# Autodesk Inventor assembly: assembly
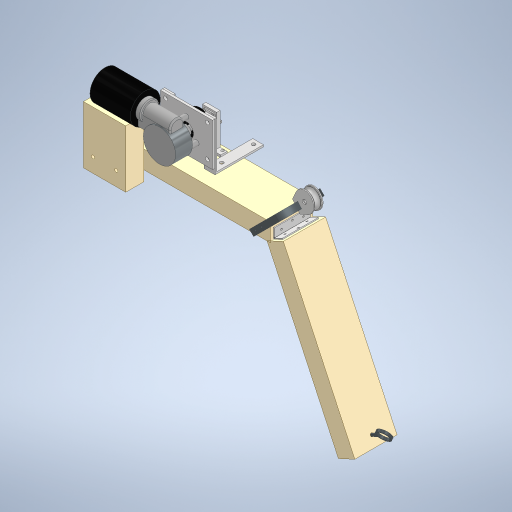
[picture p0: Inventor's stored thumbnail of the model, 512x512]
Saved by Autodesk Inventor 2024.3 (Build 283343000, 343)
## iProperties
Created: 2024-11-18
Part Number: assembly
Document SubType Name: Assembly
Designer: email
Author: email
## Documents named in this file (16)
- C:\Users\email\Desktop\Projects\Capstone\pidtest\assembly.iam
- C:\Users\email\Desktop\Projects\Capstone\pidtest\hinge.ipt
- C:\Users\email\Desktop\Projects\Capstone\pidtest\shin2x4.ipt
- C:\Users\email\Desktop\Projects\Capstone\pidtest\thigh2x4.ipt
- C:\Users\email\Desktop\Projects\Capstone\motor cad\motor.ipt
- C:\Users\email\Desktop\Projects\Capstone\pidtest\pulleybracket.ipt
- C:\Users\email\Desktop\Projects\Capstone\pidtest\hook.ipt
- C:\Users\email\Desktop\Projects\Capstone\motor cad\spool_temp.ipt
- C:\Users\email\Desktop\Projects\Capstone\pidtest\backmotormount.ipt
- C:\Users\email\Desktop\Projects\Capstone\pidtest\Lbracket.ipt
- C:\Users\email\Desktop\Projects\Capstone\pidtest\motorbracket2.ipt
- C:\Users\email\Desktop\Projects\Capstone\pidtest\pulley.ipt
- C:\Users\email\Desktop\Projects\Capstone\pidtest\pulleybearing.ipt
- C:\Users\email\Desktop\Projects\Capstone\pidtest\as5600mount.ipt
- C:\Users\email\Desktop\Projects\Capstone\pidtest\as5600.ipt
- C:\Users\email\Desktop\Projects\Capstone\pidtest\magnetholder.ipt
## Components (17 placed, 15 different names)
1. hinge:1 — Mate:1, Flush:2, Mate:33, Mate:34
2. shin2x4:1 — Mate:4, Flush:1, Mate:15, Mate:16, Mate:35
3. thigh2x4:1 — Mate:1, Flush:1, Mate:13, Mate:14, Mate:20, Mate:22, Mate:25, Mate:26, Flush:2, Mate:33, Mate:36, Mate:40, Mate:41, Mate:42, Mate:46, Mate:55, Mate:56
4. hinge:2 — Mate:4, Mate:34, Mate:35
5. motor:1 — Mate:17, Mate:18, Mate:19, Mate:30, Mate:31, Mate:32
6. pulleybracket:1 — Mate:13, Mate:14, Mate:36, Mate:37
7. hook:1 — Mate:15, Mate:16
8. spool_temp:1 — Mate:17, Mate:18, Mate:19, Mate:52, Mate:53, Mate:54
9. backmotormount:1 — Mate:20, Mate:22, Mate:40
10. Lbracket:1 — Mate:26, Mate:42, Mate:43
11. Lbracket:2 — Mate:25, Mate:41, Mate:44, Mate:45
12. motorbracket2:1 — Mate:30, Mate:31, Mate:32, Mate:43, Mate:44, Mate:45
13. pulley:1 — Mate:37, Mate:38, Mate:39
14. pulleybearing:1 — Mate:38, Mate:39
15. as5600mount:1 — Mate:46, Mate:49, Mate:50, Mate:51, Mate:55, Mate:56
16. as5600:1 — Mate:49, Mate:50, Mate:51
17. magnetholder:1 — Mate:52, Mate:53, Mate:54
## Relationships (40: Mate 38, Flush 2)
- Mate:1: hinge:1 ↔ thigh2x4:1
- Mate:4: shin2x4:1 ↔ hinge:2
- Flush:1: shin2x4:1 ↔ thigh2x4:1
- Mate:13: thigh2x4:1 ↔ pulleybracket:1
- Mate:14: thigh2x4:1 ↔ pulleybracket:1
- Mate:15: shin2x4:1 ↔ hook:1
- Mate:16 (-12.7 mm): shin2x4:1 ↔ hook:1
- Mate:17: motor:1 ↔ spool_temp:1
- Mate:18: motor:1 ↔ spool_temp:1
- Mate:19: motor:1 ↔ spool_temp:1
- Mate:20: thigh2x4:1 ↔ backmotormount:1
- Mate:22: thigh2x4:1 ↔ backmotormount:1
- Mate:25: thigh2x4:1 ↔ Lbracket:2
- Mate:26: thigh2x4:1 ↔ Lbracket:1
- Mate:30: motor:1 ↔ motorbracket2:1
- Mate:31: motor:1 ↔ motorbracket2:1
- Mate:32: motor:1 ↔ motorbracket2:1
- Flush:2 (6.35 mm): hinge:1 ↔ thigh2x4:1
- Mate:33: hinge:1 ↔ thigh2x4:1
- Mate:34: hinge:1 ↔ hinge:2
- Mate:35: shin2x4:1 ↔ hinge:2
- Mate:36: thigh2x4:1 ↔ pulleybracket:1
- Mate:37: pulleybracket:1 ↔ pulley:1
- Mate:38: pulley:1 ↔ pulleybearing:1
- Mate:39 (1.27 mm): pulley:1 ↔ pulleybearing:1
- Mate:40: thigh2x4:1 ↔ backmotormount:1
- Mate:41: thigh2x4:1 ↔ Lbracket:2
- Mate:42: thigh2x4:1 ↔ Lbracket:1
- Mate:43: Lbracket:1 ↔ motorbracket2:1
- Mate:44: Lbracket:2 ↔ motorbracket2:1
- Mate:45: Lbracket:2 ↔ motorbracket2:1
- Mate:46: thigh2x4:1 ↔ as5600mount:1
- Mate:49: as5600mount:1 ↔ as5600:1
- Mate:50: as5600mount:1 ↔ as5600:1
- Mate:51: as5600mount:1 ↔ as5600:1
- Mate:52: spool_temp:1 ↔ magnetholder:1
- Mate:53: spool_temp:1 ↔ magnetholder:1
- Mate:54: spool_temp:1 ↔ magnetholder:1
- Mate:55: thigh2x4:1 ↔ as5600mount:1
- Mate:56: thigh2x4:1 ↔ as5600mount:1
